# Autodesk Inventor assembly: bevel mechanism complete
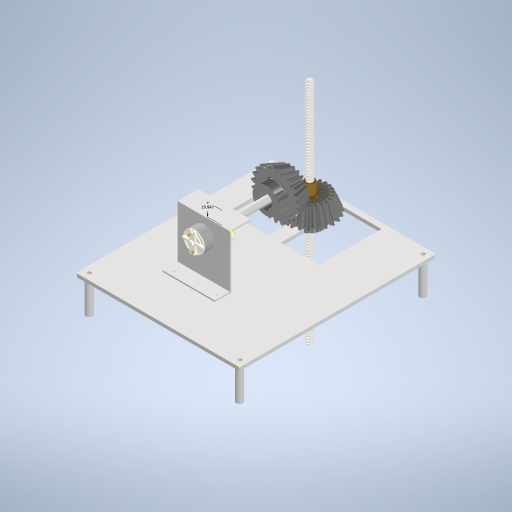
[picture p0: Inventor's stored thumbnail of the model, 512x512]
Saved by Autodesk Inventor 2024 (Build 280153000, 153)
## iProperties
Created: 2023-06-07
Part Number: bevel mechanism complete
Document SubType Name: Assembly
Designer: shraa
Author: shraa
## Documents named in this file (7)
- C:\Users\shraa\OneDrive\Documents\explo\bevel mechanism complete.iam
- C:\Users\shraa\OneDrive\Documents\explo\bevel desk.ipt
- C:\Users\shraa\OneDrive\Documents\explo\dc clamp.ipt
- C:\Users\shraa\OneDrive\Documents\explo\shaft rod.ipt
- C:\Users\shraa\Downloads\Lead Screw\8-mm lead screw.iam
- C:\Users\shraa\Downloads\DC_Motor\Inventor File\dc Motor.iam
- C:\Users\shraa\Downloads\bavel-gear-2.snapshot.1\Bavel gear.ipt
## Components (7 placed, 6 different names)
1. bevel desk:1 — Rotational:1, Rotational:2, Rotational:3, Rotational:6
2. dc clamp:1 — Rotational:1, Rotational:2, Rotational:3, Rotational:4
3. shaft rod:1 — Rotational:5, Rotational:7
4. 8-mm lead screw:1 [sub-assembly] — Rotational:8
5. dc Motor:1 [sub-assembly] — Rotational:4, Rotational:5
6. Bavel gear:1 — Rotational:7
7. Bavel gear:2 — Rotational:6, Rotational:8
## Relationships (8: RevoluteJoint 8)
- Rotational:1 [RevoluteJoint] (-3 mm): bevel desk:1 ↔ dc clamp:1
- Rotational:2 [RevoluteJoint]: bevel desk:1 ↔ dc clamp:1
- Rotational:3 [RevoluteJoint]: bevel desk:1 ↔ dc clamp:1
- Rotational:4 [RevoluteJoint]: dc clamp:1 ↔ dc Motor:1
- Rotational:5 [RevoluteJoint]: shaft rod:1 ↔ dc Motor:1
- Rotational:6 [RevoluteJoint]: bevel desk:1 ↔ Bavel gear:2
- Rotational:7 [RevoluteJoint]: shaft rod:1 ↔ Bavel gear:1
- Rotational:8 [RevoluteJoint]: 8-mm lead screw:1 ↔ Bavel gear:2
